# Autodesk Inventor assembly: wheelAssembly_1
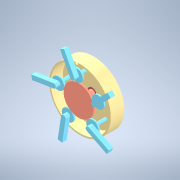
[picture p0: Inventor's stored thumbnail of the model, 180x180]
Saved by Autodesk Inventor 2020.1 (Build 241239000, 239)
## iProperties
Created: 2020-01-18
Part Number: wheelAssembly_1
Document SubType Name: Assembly
Designer: Ali
Author: Ali
## Documents named in this file (6)
- F:\Inventor_Projects\ARCS\wheelAssembly_1.iam
- F:\Inventor_Projects\ARCS\Wheel_1.ipt
- F:\Inventor_Projects\ARCS\innerGear_1.ipt
- F:\Inventor_Projects\ARCS\outerGear_2.ipt
- F:\Inventor_Projects\ARCS\bearing_1.ipt
- F:\Inventor_Projects\ARCS\Excel\New_Parameters.xlsx
## Components (8 placed, 4 different names)
1. Wheel_1:1 — Insert:1, Insert:2, Insert:3
2. innerGear_1:1 — Insert:1
3. bearing_1:1 — Insert:3
4. outerGear_2:1 — Insert:2
5. outerGear_2:2
6. outerGear_2:3
7. outerGear_2:4
8. outerGear_2:5
## Component patterns: (5 elements, first: outerGear_2:1)
## Relationships (3: Insert 3)
- Insert:1 (-69.85 mm): Wheel_1:1 ↔ innerGear_1:1
- Insert:2: Wheel_1:1 ↔ outerGear_2:1
- Insert:3: Wheel_1:1 ↔ bearing_1:1
## Named parameters: Wheel_Related_W_ = 0, W_innerDiameter = 254 mm, W_innerDepth = 50.8 mm, W_wallThickness = 6.35 mm, W_holesClearance = 0.254 mm, W_outerGearHoleDiameter = 13.208 mm, W_innerGearHoleDiameter = 38.608 mm, TempSpotReserved7 = 0 mm, TempSpotReserved8 = 0 mm, TempSpotReserved9 = 0 mm, TempSpotReserved10 = 0 mm, TempSpotReserved11 = 0 mm, TempSpotReserved12 = 0 mm, TempSpotReserved13 = 0 mm, TempSpotReserved14 = 0 mm, TempSpotReserved15 = 0 mm, TempSpotReserved16 = 0 mm, TempSpotReserved17 = 0 mm, TempSpotReserved18 = 0 mm, TempSpotReserved19 = 0 mm, TempSpotReserved20 = 0 mm, Inner_Gear_Related_IG_ = 0, IG_shaftDiameter = 25.4 mm, IG_gearDiameter = 127 mm, IG_shaftLength = 127 mm, IG_gearThickness = 6.35 mm, TempSpotReserved25 = 0 mm, TempSpotReserved26 = 0 mm, TempSpotReserved27 = 0 mm, TempSpotReserved28 = 0 mm, TempSpotReserved29 = 0 mm, TempSpotReserved30 = 0 mm, TempSpotReserved31 = 0 mm, TempSpotReserved32 = 0 mm, TempSpotReserved33 = 0 mm, TempSpotReserved34 = 0 mm, TempSpotReserved35 = 0 mm, TempSpotReserved36 = 0 mm, TempSpotReserved37 = 0 mm, TempSpotReserved38 = 0 mm, TempSpotReserved39 = 0 mm, TempSpotReserved40 = 0 mm, Outer_Gear_Related_OG_ = 0, OG_distanceFromCenter = 88.9 mm, OG_shaftDiameter = 12.7 mm, OG_gearDiameter = 50.8 mm, OG_numberOfGears = 5, OG_shaftLength = 57.15 mm, OG_gearThickness = 6.35 mm, TempSpotReserved47 = 0 mm, TempSpotReserved48 = 0 mm, TempSpotReserved49 = 0 mm, TempSpotReserved50 = 0 mm, TempSpotReserved51 = 0 mm, TempSpotReserved52 = 0 mm, TempSpotReserved53 = 0 mm, TempSpotReserved54 = 0 mm, TempSpotReserved55 = 0 mm, TempSpotReserved56 = 0 mm, TempSpotReserved57 = 0 mm, TempSpotReserved58 = 0 mm, TempSpotReserved59 = 0 mm, TempSpotReserved60 = 0 mm, Leg_Extensions_Related_LE_ = 0, LE_baseDiameter = 19.05 mm, LE_maxLength = 93.92488 mm, LE_thickness = 19.05 mm, IG_ratioToOuterGear = 2.5, B_bearingThickness = 6.35 mm, TempSpotReserved43 = 0 mm, TempSpotReserved45 = 0 mm, Thisisatest = 25.4 mm, TempSpotReserved46 = 0 mm, TempSpotReserved44 = 0 mm, LE_offsetAboveOuterGear = 0 mm, Bearing_Related_B_ = 0, TempSpotReserved42 = 0 mm
